# Autodesk Inventor assembly: RobotTry3
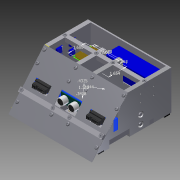
[picture p0: Inventor's stored thumbnail of the model, 180x180]
Saved by Autodesk Inventor 2012 (Build 160160000, 160)
## iProperties
Created: 2012-04-08
Part Number: RobotTry3
Document SubType Name: Assembly
Designer: admin
Mass: 2820.16 g
Surface Area: 4873.11 cm^2
Volume: 937.85 cm^3
Density: 3.00704 g/cm^3
Author: admin
## Documents named in this file (55)
- C:\Users\Admin\Documents\Inventor\SumoJaime2012\RobotTry3.iam
- C:\Users\Admin\Documents\Inventor\SumoJaime2012\BaneBotWheel.iam
- C:\Users\Admin\Documents\Inventor\SumoJaime2012\Design Accelerator\Spur Gear11.ipt
- C:\Users\Admin\Documents\Inventor\SumoJaime2012\Design Accelerator\Shaft1.iam
- C:\Users\Admin\Documents\Inventor\SumoJaime2012\Imported Components\s1066z-032s014\s1066z-032s014-2.ipt
- C:\Users\Admin\Documents\Inventor\SumoJaime2012\Imported Components\s1066z-032s036\s1066z-032s036.ipt
- C:\Users\Admin\Documents\Inventor\SumoJaime2012\Imported Components\s1066z-032s075\s1066z-032s075-2.ipt
- C:\Users\Admin\Documents\Inventor\SumoJaime2012\Imported Components\s1066z-032s075\ShaftStraight.ipt
- C:\Users\Admin\Documents\Inventor\SumoJaime2012\MabuchiRS550.ipt
- C:\Users\Admin\Documents\Inventor\SumoJaime2012\Chassis Right3.ipt
- C:\Users\Admin\Documents\Inventor\SumoJaime2012\Inside Chassis3.ipt
- C:\Users\Admin\Documents\Inventor\SumoJaime2012\Bearing57155K323.ipt
- C:\Users\Admin\Documents\Inventor\SumoJaime2012\Turnigy2200mAh4S40C.ipt
- C:\Users\Admin\Documents\Inventor\SumoJaime2012\Imported Components\97633A130\97633A130.ipt
- C:\Users\Admin\Documents\Inventor\SumoJaime2012\BaneBotWheel_MIR2.iam
- C:\Users\Admin\Documents\Inventor\SumoJaime2012\Design Accelerator\Spur Gear11_MIR2.ipt
- C:\Users\Admin\Documents\Inventor\SumoJaime2012\Design Accelerator\Shaft1_MIR2.iam
- C:\Users\Admin\Documents\Inventor\SumoJaime2012\Imported Components\s1066z-032s014\s1066z-032s014-2_MIR2.ipt
- C:\Users\Admin\Documents\Inventor\SumoJaime2012\Imported Components\s1066z-032s036\s1066z-032s036_MIR2.ipt
- C:\Users\Admin\Documents\Inventor\SumoJaime2012\Imported Components\s1066z-032s075\s1066z-032s075-2_MIR2.ipt
- C:\Users\Admin\Documents\Inventor\SumoJaime2012\Imported Components\s1066z-032s075\ShaftStraight_MIR2.ipt
- C:\Users\Admin\Documents\Inventor\SumoJaime2012\MabuchiRS550_MIR1.ipt
- C:\Users\Admin\Documents\Inventor\SumoJaime2012\Chassis Right3_MIR.ipt
- C:\Users\Admin\Documents\Inventor\SumoJaime2012\Inside Chassis3_MIR.ipt
- C:\Users\Admin\Documents\Inventor\SumoJaime2012\Bearing57155K323_MIR1.ipt
- C:\Users\Admin\Documents\Inventor\SumoJaime2012\Imported Components\97633A130\97633A130_MIR.ipt
- C:\Users\Admin\Documents\Inventor\SumoJaime2012\MagnetAssembly.iam
- C:\Users\Admin\Documents\Inventor\SumoJaime2012\Chassis Back.ipt
- C:\Users\Admin\Documents\Inventor\SumoJaime2012\ChassisFrontPlate.ipt
- C:\Users\Admin\Documents\Inventor\SumoJaime2012\Battery Board.ipt
- C:\Users\Admin\Documents\Inventor\SumoJaime2012\Parallax Ping Sensor.iam
- C:\Users\Admin\Documents\Inventor\SumoJaime2012\QTR1A.ipt
- C:\Users\Admin\Documents\Inventor\SumoJaime2012\Sharp GP2Y0 Sensor.iam
- C:\Users\Admin\Documents\Inventor\SumoJaime2012\SensorBar.ipt
- C:\Users\Admin\Documents\Inventor\SumoJaime2012\Blade.ipt
- C:\Users\Admin\Documents\Inventor\SumoJaime2012\Protector.ipt
- C:\Users\Admin\Documents\Inventor\SumoJaime2012\NMOS.ipt
- C:\Users\Admin\Documents\Inventor\SumoJaime2012\SupportBar.ipt
- C:\Users\Admin\Documents\Inventor\SumoJaime2012\RobotTry3\Design Accelerator\Bolted Connection2.iam
- C:\Users\Admin\Documents\Inventor\SumoJaime2012\RobotTry3\Design Accelerator\Bolted Connection3.iam
- C:\Users\Admin\Documents\Inventor\SumoJaime2012\RobotTry3\Design Accelerator\Bolted Connection4.iam
- C:\Users\Admin\Documents\Inventor\SumoJaime2012\RobotTry3\Design Accelerator\Bolted Connection5.iam
- C:\Users\Admin\Documents\Inventor\SumoJaime2012\RobotTry3\Design Accelerator\Bolted Connection6.iam
- C:\Users\Admin\Documents\Inventor\SumoJaime2012\RobotTry3\Design Accelerator\Bolted Connection7.iam
- C:\Users\Admin\Documents\Inventor\SumoJaime2012\RobotTry3\Design Accelerator\Bolted Connection8.iam
- C:\Users\Admin\Documents\Inventor\SumoJaime2012\RobotTry3\Design Accelerator\Bolted Connection9.iam
- C:\Users\Admin\Documents\Inventor\SumoJaime2012\RobotTry3\Design Accelerator\Bolted Connection10.iam
- C:\Users\Admin\Documents\Inventor\SumoJaime2012\RobotTry3\Design Accelerator\Bolted Connection11.iam
- C:\Users\Admin\Documents\Inventor\SumoJaime2012\RobotTry3\Design Accelerator\Bolted Connection12.iam
- C:\Users\Admin\Documents\Inventor\SumoJaime2012\RobotTry3\Design Accelerator\Bolted Connection13.iam
- C:\Users\Admin\Documents\Inventor\SumoJaime2012\RobotTry3\Design Accelerator\Bolted Connection14.iam
- C:\Users\Admin\Documents\Inventor\SumoJaime2012\RobotTry3\Design Accelerator\Bolted Connection15.iam
- C:\Users\Admin\Documents\Inventor\SumoJaime2012\RobotTry3\Design Accelerator\Bolted Connection16.iam
- C:\Users\Admin\Documents\Inventor\SumoJaime2012\ElectronicsBoard.ipt
- C:\Users\Admin\Documents\Inventor\SumoJaime2012\RobotTry3\Design Accelerator\Bolted Connection17.iam
## Components (74 placed, 39 different names)
1. BaneBotWheel:1 [sub-assembly] — Mate:4, Mate:5, Mate:6, Mate:8, Flush:7, Tangent:3
2. Spur Gear1:1 — Tangent:2, Mate:9, Mate:10
3. Shaft:2 [sub-assembly] — Mate:5, Mate:6, Mate:7, Mate:8, Flush:3, Flush:7, Flush:9, Mate:19, Mate:20
4. s1066z-032s014-2:1 — Tangent:1, Mate:1, Mate:2, Flush:5, Flush:10
5. s1066z-032s036:1 — Tangent:1, Mate:4, Mate:7, Flush:10
6. s1066z-032s075-2:1 — Mate:1, Tangent:2, Mate:3, Flush:8, Mate:15
7. ShaftStraight:1 — Mate:2, Mate:3, Flush:3, Flush:5, Flush:8, Angle:4, Mate:17, Mate:18, Flush:14, Mate:26, Mate:27, Mate:28, Mate:29, Mate:59
8. MabuchiRS550:1 — Mate:9, Mate:10, Mate:14, Angle:5, Mate:16
9. Chassis Right3:1 — Mate:11, Mate:12, Mate:13, Flush:11, Flush:12, Flush:13, Mate:24, Mate:25, Flush:14, Flush:28, Mate:62, Flush:30, Mate:66, Flush:32, Flush:33, Mate:78, Mate:79, Mate:80, Flush:37, Flush:40, Flush:42, Mate:87, Mate:91, Flush:46, Flush:47, Mate:92, Mate:93, Mate:94, Mate:95, Flush:57, Flush:58, Flush:59, Mate:117, Mate:144
10. Inside Chassis3:1 — Mate:14, Mate:15, Flush:9, Tangent:3, Mate:16, Mate:21, Mate:22, Mate:23, Flush:11, Flush:12, Flush:13, Flush:25, Flush:26, Flush:29, Mate:72, Mate:100, Mate:101, Mate:102
11. Bearing57155K323:1 — Mate:19, Mate:25
12. Bearing57155K323:2 — Mate:18, Mate:23
13. Bearing57155K323:3 — Mate:20, Mate:21, Mate:22
14. Bearing57155K323:4 — Mate:17, Mate:24
15. Turnigy2200mAh4S40C:1 — Mate:68, Mate:69, Mate:77
16. 97633A130:1 — Mate:26, Mate:27
17. 97633A130:2 — Mate:28, Mate:29
18. BaneBotWheel_MIR2:1 [sub-assembly] — Flush:15, Mate:30, Mate:31, Mate:32, Mate:34, Tangent:6
19. Spur Gear11_MIR2:1 — Tangent:5, Mate:38, Mate:39
20. Shaft1_MIR2:1 [sub-assembly] — Flush:15, Mate:30, Mate:31, Mate:32, Mate:33, Flush:19, Flush:24, Mate:47, Mate:52
21. s1066z-032s014-2_MIR2:1 — Flush:16, Tangent:4, Mate:35, Flush:18, Mate:37
22. s1066z-032s036_MIR2:1 — Flush:16, Mate:33, Mate:34, Tangent:4
23. s1066z-032s075-2_MIR2:1 — Tangent:5, Mate:35, Flush:17, Mate:36, Mate:44
24. ShaftStraight_MIR2:1 — Flush:17, Flush:18, Flush:19, Mate:36, Mate:37, Flush:20, Mate:49, Mate:54, Mate:55, Mate:56, Mate:57, Mate:58, Mate:59
25. MabuchiRS550_MIR1:1 — Mate:38, Mate:39, Mate:43, Mate:45
26. Chassis Right3_MIR:1 — Flush:20, Flush:21, Flush:22, Flush:23, Mate:46, Mate:53, Flush:27, Flush:31, Mate:64, Mate:70, Mate:71, Mate:77, Mate:81, Mate:82, Mate:88, Flush:43, Mate:90, Flush:44, Flush:45, Mate:96, Mate:97, Mate:98, Mate:99, Flush:56, Flush:63, Mate:109, Mate:110, Mate:111, Mate:112, Mate:118
27. Inside Chassis3_MIR:1 — Flush:21, Flush:22, Flush:23, Mate:43, Tangent:6, Flush:24, Mate:44, Mate:45, Mate:48, Mate:50, Mate:51, Flush:25, Flush:26, Mate:63
28. Bearing57155K323_MIR1:1 — Mate:46, Mate:47
29. Bearing57155K323_MIR1:2 — Mate:48, Mate:49
30. Bearing57155K323_MIR1:3 — Mate:50, Mate:51, Mate:52
31. Bearing57155K323_MIR1:4 — Mate:53, Mate:54
32. 97633A130_MIR:1 — Mate:55, Mate:56
33. 97633A130_MIR:2 — Mate:57, Mate:58
34. MagnetAssembly:1 [sub-assembly] — Flush:27, Flush:28, Mate:70, Mate:71, Mate:115, Mate:116, Mate:125, Mate:126, Mate:127, Mate:128, Mate:129, Mate:130, Mate:131, Mate:132, Mate:133, Mate:134, Mate:135, Mate:136, Mate:137, Mate:138, Mate:139, Mate:140
35. Chassis Back:1 — Mate:62, Flush:29, Flush:30, Mate:67, Mate:69, Flush:32, Angle:6, Mate:113, Mate:114, Mate:143
36. ChassisFrontPlate:1 — Mate:63, Flush:31, Mate:64, Mate:83, Mate:84
37. Battery Board:1 — Mate:66, Mate:67, Mate:68, Mate:72, Mate:105, Mate:141, Mate:147, Mate:148
38. Parallax Ping Sensor:1 [sub-assembly] — Flush:34, Mate:74, Mate:82
39. QTR1A:1 — Flush:42, Mate:87, Mate:117
40. QTR1A:2 — Mate:91, Flush:46, Flush:47
41. QTR1A:3 — Mate:88, Flush:43, Mate:118
42. QTR1A:4 — Mate:90, Flush:44, Flush:45
43. Sharp GP2Y0 Sensor:1 [sub-assembly] — Flush:36, Mate:76, Mate:81
44. Sharp GP2Y0 Sensor:2 [sub-assembly] — Flush:35, Mate:75, Mate:80
45. SensorBar:1 — Flush:33, Angle:6, Flush:34, Mate:74, Flush:35, Mate:75, Flush:36, Mate:76, Mate:78, Mate:79
46. Blade:1 — Mate:83, Mate:84, Flush:37, Flush:39, Mate:85, Mate:123, Mate:124
47. Protector:1 — Flush:39, Mate:85, Flush:40, Mate:119, Mate:120
48. NMOS:1 — Mate:99, Mate:112, Flush:64
49. NMOS:2 — Mate:98, Mate:111, Flush:65, Flush:66
50. NMOS:3 — Mate:96, Mate:110, Flush:65
51. NMOS:4 — Mate:97, Flush:63, Mate:109, Flush:64, Flush:66
52. NMOS:5 — Mate:92, Flush:62, Mate:108
53. NMOS:6 — Mate:93, Flush:60, Mate:106, Flush:62, Mate:108
54. NMOS:7 — Mate:94, Flush:61, Mate:107
55. NMOS:8 — Mate:95, Flush:59, Mate:105, Flush:60, Mate:106, Flush:61, Mate:107
56. SupportBar:1 — Flush:56, Mate:100, Flush:57, Mate:103, Mate:104
57. SupportBar:2 — Mate:101, Mate:102, Flush:58, Mate:121, Mate:122
58. Bolted Connection:1 [sub-assembly] — Mate:103, Mate:104
59. Bolted Connection:2 [sub-assembly] — Mate:113, Mate:114
60. Bolted Connection:3 [sub-assembly] — Mate:115, Mate:116
61. Bolted Connection:4 [sub-assembly] — Mate:119, Mate:120
62. Bolted Connection:5 [sub-assembly] — Mate:121, Mate:122
63. Bolted Connection:6 [sub-assembly] — Mate:123, Mate:124
64. Bolted Connection:7 [sub-assembly]
65. Bolted Connection:8 [sub-assembly] — Mate:125, Mate:126
66. Bolted Connection:9 [sub-assembly] — Mate:127, Mate:128
67. Bolted Connection:10 [sub-assembly] — Mate:129, Mate:130
68. Bolted Connection:11 [sub-assembly] — Mate:131, Mate:132
69. Bolted Connection:12 [sub-assembly] — Mate:133, Mate:134
70. Bolted Connection:13 [sub-assembly] — Mate:135, Mate:136
71. Bolted Connection:14 [sub-assembly] — Mate:137, Mate:138
72. Bolted Connection:15 [sub-assembly] — Mate:139, Mate:140
73. ElectronicsBoard:2 — Mate:141, Mate:143, Mate:144
74. Bolted Connection:16 [sub-assembly] — Mate:147, Mate:148
## Relationships (197: Mate 136, Flush 52, Tangent 6, Angle 3)
- Tangent:1 (0.0508 mm): s1066z-032s014-2:1 ↔ s1066z-032s036:1
- Mate:1: s1066z-032s014-2:1 ↔ s1066z-032s075-2:1
- Tangent:2 (0.0508 mm): Spur Gear1:1 ↔ s1066z-032s075-2:1
- Mate:2: s1066z-032s014-2:1 ↔ ShaftStraight:1
- Mate:3: s1066z-032s075-2:1 ↔ ShaftStraight:1
- Mate:4: BaneBotWheel:1 ↔ s1066z-032s036:1
- Mate:5: BaneBotWheel:1 ↔ Shaft:2
- Mate:6: BaneBotWheel:1 ↔ Shaft:2
- Mate:7: Shaft:2 ↔ s1066z-032s036:1
- Mate:8: BaneBotWheel:1 ↔ Shaft:2
- Mate:9: Spur Gear1:1 ↔ MabuchiRS550:1
- Mate:10: Spur Gear1:1 ↔ MabuchiRS550:1
- Mate:11: Chassis Right3:1
- Mate:12: Chassis Right3:1
- Mate:13: Chassis Right3:1
- Mate:14: MabuchiRS550:1 ↔ Inside Chassis3:1
- Flush:3: Shaft:2 ↔ ShaftStraight:1
- Flush:5 (25.4 mm): s1066z-032s014-2:1 ↔ ShaftStraight:1
- Flush:7 (2.54 mm): BaneBotWheel:1 ↔ Shaft:2
- Flush:8: s1066z-032s075-2:1 ↔ ShaftStraight:1
- Mate:15 (2.54 mm): s1066z-032s075-2:1 ↔ Inside Chassis3:1
- Flush:9: Shaft:2 ↔ Inside Chassis3:1
- Angle:4 (0 deg): ShaftStraight:1
- Tangent:3 (-5.08 mm): BaneBotWheel:1 ↔ Inside Chassis3:1
- Angle:5 (0 deg): MabuchiRS550:1
- Flush:10: s1066z-032s014-2:1 ↔ s1066z-032s036:1
- Mate:16: MabuchiRS550:1 ↔ Inside Chassis3:1
- Mate:17: ShaftStraight:1 ↔ Bearing57155K323:4
- Mate:18: ShaftStraight:1 ↔ Bearing57155K323:2
- Mate:19: Shaft:2 ↔ Bearing57155K323:1
- Mate:20: Shaft:2 ↔ Bearing57155K323:3
- Mate:21: Inside Chassis3:1 ↔ Bearing57155K323:3
- Mate:22: Inside Chassis3:1 ↔ Bearing57155K323:3
- Mate:23: Inside Chassis3:1 ↔ Bearing57155K323:2
- Flush:11: Chassis Right3:1 ↔ Inside Chassis3:1
- Flush:12: Chassis Right3:1 ↔ Inside Chassis3:1
- Flush:13: Chassis Right3:1 ↔ Inside Chassis3:1
- Mate:24: Chassis Right3:1 ↔ Bearing57155K323:4
- Mate:25: Chassis Right3:1 ↔ Bearing57155K323:1
- Flush:14: ShaftStraight:1 ↔ Chassis Right3:1
- Mate:26: ShaftStraight:1 ↔ 97633A130:1
- Mate:27: ShaftStraight:1 ↔ 97633A130:1
- Mate:28: ShaftStraight:1 ↔ 97633A130:2
- Mate:29: ShaftStraight:1 ↔ 97633A130:2
- Flush:15 (2.54 mm): BaneBotWheel_MIR2:1 ↔ Shaft1_MIR2:1
- Mate:30: BaneBotWheel_MIR2:1 ↔ Shaft1_MIR2:1
- Mate:31: BaneBotWheel_MIR2:1 ↔ Shaft1_MIR2:1
- Mate:32: BaneBotWheel_MIR2:1 ↔ Shaft1_MIR2:1
- Flush:16: s1066z-032s014-2_MIR2:1 ↔ s1066z-032s036_MIR2:1
- Mate:33: Shaft1_MIR2:1 ↔ s1066z-032s036_MIR2:1
- Mate:34: BaneBotWheel_MIR2:1 ↔ s1066z-032s036_MIR2:1
- Tangent:4 (0.0508 mm): s1066z-032s014-2_MIR2:1 ↔ s1066z-032s036_MIR2:1
- Tangent:5 (0.0508 mm): Spur Gear11_MIR2:1 ↔ s1066z-032s075-2_MIR2:1
- Mate:35: s1066z-032s014-2_MIR2:1 ↔ s1066z-032s075-2_MIR2:1
- Flush:17: s1066z-032s075-2_MIR2:1 ↔ ShaftStraight_MIR2:1
- Flush:18 (25.4 mm): s1066z-032s014-2_MIR2:1 ↔ ShaftStraight_MIR2:1
- Flush:19: Shaft1_MIR2:1 ↔ ShaftStraight_MIR2:1
- Mate:36: s1066z-032s075-2_MIR2:1 ↔ ShaftStraight_MIR2:1
- Mate:37: s1066z-032s014-2_MIR2:1 ↔ ShaftStraight_MIR2:1
- Mate:38: Spur Gear11_MIR2:1 ↔ MabuchiRS550_MIR1:1
- Mate:39: Spur Gear11_MIR2:1 ↔ MabuchiRS550_MIR1:1
- Flush:20: ShaftStraight_MIR2:1 ↔ Chassis Right3_MIR:1
- Flush:21: Chassis Right3_MIR:1 ↔ Inside Chassis3_MIR:1
- Flush:22: Chassis Right3_MIR:1 ↔ Inside Chassis3_MIR:1
- Flush:23: Chassis Right3_MIR:1 ↔ Inside Chassis3_MIR:1
- Mate:43: MabuchiRS550_MIR1:1 ↔ Inside Chassis3_MIR:1
- Tangent:6 (-5.08 mm): BaneBotWheel_MIR2:1 ↔ Inside Chassis3_MIR:1
- Flush:24: Shaft1_MIR2:1 ↔ Inside Chassis3_MIR:1
- Mate:44 (2.54 mm): s1066z-032s075-2_MIR2:1 ↔ Inside Chassis3_MIR:1
- Mate:45: MabuchiRS550_MIR1:1 ↔ Inside Chassis3_MIR:1
- Mate:46: Chassis Right3_MIR:1 ↔ Bearing57155K323_MIR1:1
- Mate:47: Shaft1_MIR2:1 ↔ Bearing57155K323_MIR1:1
- Mate:48: Inside Chassis3_MIR:1 ↔ Bearing57155K323_MIR1:2
- Mate:49: ShaftStraight_MIR2:1 ↔ Bearing57155K323_MIR1:2
- Mate:50: Inside Chassis3_MIR:1 ↔ Bearing57155K323_MIR1:3
- Mate:51: Inside Chassis3_MIR:1 ↔ Bearing57155K323_MIR1:3
- Mate:52: Shaft1_MIR2:1 ↔ Bearing57155K323_MIR1:3
- Mate:53: Chassis Right3_MIR:1 ↔ Bearing57155K323_MIR1:4
- Mate:54: ShaftStraight_MIR2:1 ↔ Bearing57155K323_MIR1:4
- Mate:55: ShaftStraight_MIR2:1 ↔ 97633A130_MIR:1
- Mate:56: ShaftStraight_MIR2:1 ↔ 97633A130_MIR:1
- Mate:57: ShaftStraight_MIR2:1 ↔ 97633A130_MIR:2
- Mate:58: ShaftStraight_MIR2:1 ↔ 97633A130_MIR:2
- Flush:25: Inside Chassis3:1 ↔ Inside Chassis3_MIR:1
- Flush:26: Inside Chassis3:1 ↔ Inside Chassis3_MIR:1
- Mate:59 (5.08 mm): ShaftStraight:1 ↔ ShaftStraight_MIR2:1
- Flush:27: Chassis Right3_MIR:1 ↔ MagnetAssembly:1
- Flush:28: Chassis Right3:1 ↔ MagnetAssembly:1
- Mate:62: Chassis Right3:1 ↔ Chassis Back:1
- Flush:29: Inside Chassis3:1 ↔ Chassis Back:1
- Flush:30: Chassis Right3:1 ↔ Chassis Back:1
- Mate:63: Inside Chassis3_MIR:1 ↔ ChassisFrontPlate:1
- Flush:31: Chassis Right3_MIR:1 ↔ ChassisFrontPlate:1
- Mate:64: Chassis Right3_MIR:1 ↔ ChassisFrontPlate:1
- Mate:66: Chassis Right3:1 ↔ Battery Board:1
- Mate:67: Chassis Back:1 ↔ Battery Board:1
- Mate:68: Turnigy2200mAh4S40C:1 ↔ Battery Board:1
- Mate:69: Turnigy2200mAh4S40C:1 ↔ Chassis Back:1
- Mate:70 (0.0508 mm): Chassis Right3_MIR:1 ↔ MagnetAssembly:1
- Mate:71: Chassis Right3_MIR:1 ↔ MagnetAssembly:1
- Mate:72: Inside Chassis3:1 ↔ Battery Board:1
- Flush:32: Chassis Right3:1 ↔ Chassis Back:1
- Flush:33: Chassis Right3:1 ↔ SensorBar:1
- Angle:6 (180 deg): Chassis Back:1 ↔ SensorBar:1
- Flush:34: Parallax Ping Sensor:1 ↔ SensorBar:1
- Mate:74: Parallax Ping Sensor:1 ↔ SensorBar:1
- Flush:35 (-2.54 mm): Sharp GP2Y0 Sensor:2 ↔ SensorBar:1
- Mate:75: Sharp GP2Y0 Sensor:2 ↔ SensorBar:1
- Flush:36 (2.54 mm): Sharp GP2Y0 Sensor:1 ↔ SensorBar:1
- Mate:76: Sharp GP2Y0 Sensor:1 ↔ SensorBar:1
- Mate:77: Turnigy2200mAh4S40C:1 ↔ Chassis Right3_MIR:1
- Mate:78: Chassis Right3:1 ↔ SensorBar:1
- Mate:79: Chassis Right3:1 ↔ SensorBar:1
- Mate:80 (10.16 mm): Chassis Right3:1 ↔ Sharp GP2Y0 Sensor:2
- Mate:81 (10.16 mm): Chassis Right3_MIR:1 ↔ Sharp GP2Y0 Sensor:1
- Mate:82 (65.405 mm): Chassis Right3_MIR:1 ↔ Parallax Ping Sensor:1
- Mate:83: ChassisFrontPlate:1 ↔ Blade:1
- Mate:84 (-8.89 mm): ChassisFrontPlate:1 ↔ Blade:1
- Flush:37: Chassis Right3:1 ↔ Blade:1
- Flush:39: Blade:1 ↔ Protector:1
- Mate:85: Blade:1 ↔ Protector:1
- Flush:40: Chassis Right3:1 ↔ Protector:1
- Flush:42: Chassis Right3:1 ↔ QTR1A:1
- Mate:87: Chassis Right3:1 ↔ QTR1A:1
- Mate:88: Chassis Right3_MIR:1 ↔ QTR1A:3
- Flush:43: Chassis Right3_MIR:1 ↔ QTR1A:3
- Mate:90: Chassis Right3_MIR:1 ↔ QTR1A:4
- Flush:44: Chassis Right3_MIR:1 ↔ QTR1A:4
- Flush:45: Chassis Right3_MIR:1 ↔ QTR1A:4
- Mate:91: Chassis Right3:1 ↔ QTR1A:2
- Flush:46: Chassis Right3:1 ↔ QTR1A:2
- Flush:47: Chassis Right3:1 ↔ QTR1A:2
- Mate:92: Chassis Right3:1 ↔ NMOS:5
- Mate:93: Chassis Right3:1 ↔ NMOS:6
- Mate:94: Chassis Right3:1 ↔ NMOS:7
- Mate:95: Chassis Right3:1 ↔ NMOS:8
- Mate:96: Chassis Right3_MIR:1 ↔ NMOS:3
- Mate:97: Chassis Right3_MIR:1 ↔ NMOS:4
- Mate:98: Chassis Right3_MIR:1 ↔ NMOS:2
- Mate:99: Chassis Right3_MIR:1 ↔ NMOS:1
- Flush:56: Chassis Right3_MIR:1 ↔ SupportBar:1
- Mate:100: Inside Chassis3:1 ↔ SupportBar:1
- Flush:57: Chassis Right3:1 ↔ SupportBar:1
- Mate:101: Inside Chassis3:1 ↔ SupportBar:2
- Mate:102: Inside Chassis3:1 ↔ SupportBar:2
- Flush:58: Chassis Right3:1 ↔ SupportBar:2
- Mate:103: SupportBar:1 ↔ Bolted Connection:1
- Mate:104: SupportBar:1 ↔ Bolted Connection:1
- Flush:59 (12.065 mm): Chassis Right3:1 ↔ NMOS:8
- Mate:105: Battery Board:1 ↔ NMOS:8
- Flush:60: NMOS:6 ↔ NMOS:8
- Mate:106 (7.62 mm): NMOS:6 ↔ NMOS:8
- Flush:61: NMOS:7 ↔ NMOS:8
- Mate:107 (15.24 mm): NMOS:7 ↔ NMOS:8
- Flush:62: NMOS:5 ↔ NMOS:6
- Mate:108 (15.24 mm): NMOS:5 ↔ NMOS:6
- Flush:63 (12.065 mm): Chassis Right3_MIR:1 ↔ NMOS:4
- Mate:109: Chassis Right3_MIR:1 ↔ NMOS:4
- Mate:110: Chassis Right3_MIR:1 ↔ NMOS:3
- Mate:111: Chassis Right3_MIR:1 ↔ NMOS:2
- Mate:112: Chassis Right3_MIR:1 ↔ NMOS:1
- Flush:64: NMOS:1 ↔ NMOS:4
- Flush:65: NMOS:2 ↔ NMOS:3
- Flush:66: NMOS:2 ↔ NMOS:4
- Mate:113: Chassis Back:1 ↔ Bolted Connection:2
- Mate:114: Chassis Back:1 ↔ Bolted Connection:2
- Mate:115: MagnetAssembly:1 ↔ Bolted Connection:3
- Mate:116: MagnetAssembly:1 ↔ Bolted Connection:3
- Mate:117: Chassis Right3:1 ↔ QTR1A:1
- Mate:118: Chassis Right3_MIR:1 ↔ QTR1A:3
- Mate:119: Protector:1 ↔ Bolted Connection:4
- Mate:120: Protector:1 ↔ Bolted Connection:4
- Mate:121: SupportBar:2 ↔ Bolted Connection:5
- Mate:122: SupportBar:2 ↔ Bolted Connection:5
- Mate:123: Blade:1 ↔ Bolted Connection:6
- Mate:124: Blade:1 ↔ Bolted Connection:6
- Mate:125: MagnetAssembly:1 ↔ Bolted Connection:8
- Mate:126: MagnetAssembly:1 ↔ Bolted Connection:8
- Mate:127: MagnetAssembly:1 ↔ Bolted Connection:9
- Mate:128: MagnetAssembly:1 ↔ Bolted Connection:9
- Mate:129: MagnetAssembly:1 ↔ Bolted Connection:10
- Mate:130: MagnetAssembly:1 ↔ Bolted Connection:10
- Mate:131: MagnetAssembly:1 ↔ Bolted Connection:11
- Mate:132: MagnetAssembly:1 ↔ Bolted Connection:11
- Mate:133: MagnetAssembly:1 ↔ Bolted Connection:12
- Mate:134: MagnetAssembly:1 ↔ Bolted Connection:12
- Mate:135: MagnetAssembly:1 ↔ Bolted Connection:13
- Mate:136: MagnetAssembly:1 ↔ Bolted Connection:13
- Mate:137: MagnetAssembly:1 ↔ Bolted Connection:14
- Mate:138: MagnetAssembly:1 ↔ Bolted Connection:14
- Mate:139: MagnetAssembly:1 ↔ Bolted Connection:15
- Mate:140: MagnetAssembly:1 ↔ Bolted Connection:15
- Mate:141: Battery Board:1 ↔ ElectronicsBoard:2
- Mate:143 (0.254 mm): Chassis Back:1 ↔ ElectronicsBoard:2
- Mate:144: Chassis Right3:1 ↔ ElectronicsBoard:2
- Mate:147: Battery Board:1 ↔ Bolted Connection:16
- Mate:148: Battery Board:1 ↔ Bolted Connection:16
